# Autodesk Inventor assembly: ArmPower
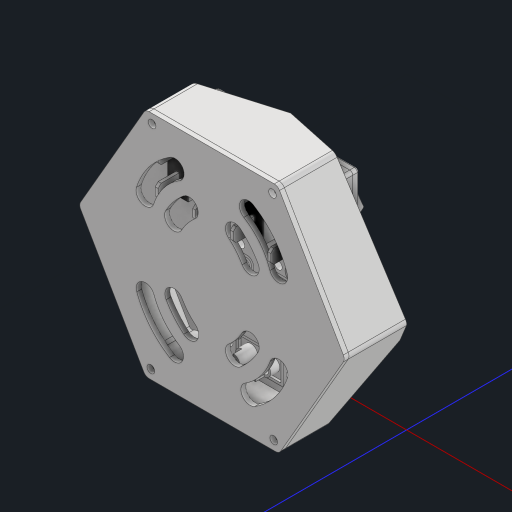
[picture p0: Inventor's stored thumbnail of the model, 512x512]
Saved by Autodesk Inventor 2023 (Build 270158000, 158)
## iProperties
Created: 2023-12-09
Part Number: ArmPower
Document SubType Name: Assembly
Designer: valer
Author: valer
## Documents named in this file (5)
- C:\Users\valer\Desktop\str1ker\cad\ArmPower.iam
- C:\Users\valer\Desktop\str1ker\cad\ArmPowerBoardWithControls.ipt
- C:\Users\valer\Desktop\str1ker\cad\ArmPowerBoardWithControlsLid.ipt
- C:\Users\valer\Desktop\str1ker\cad\external\XT-60EW-M.ipt
- C:\Users\valer\Desktop\str1ker\cad\external\ESwitchRD1.ipt
## Components (11 placed, 4 different names)
1. ArmPowerBoardWithControls:1 — Mate:1, Mate:2, Mate:3, Mate:4, Mate:5, Mate:6, Mate:7, Mate:8, Mate:9, Mate:10, Mate:11, Mate:12, Mate:13, Mate:14, Mate:15, Mate:16, Mate:17, Mate:18, Mate:19, Mate:20, Mate:21, Mate:22, Mate:23, Mate:24, Mate:25, Mate:26, Mate:27
2. ArmPowerBoardWithControlsLid:1 — Mate:1, Mate:2, Mate:3
3. XT-60EW-M:1 — Mate:4, Mate:5, Mate:6, Flush:1
4. ESwitchRD1:1 — Mate:7, Mate:8, Mate:9
5. ESwitchRD1:2 — Mate:10, Mate:11, Mate:12
6. ESwitchRD1:3 — Mate:13, Mate:14, Mate:15
7. ESwitchRD1:4 — Mate:16, Mate:17, Mate:18
8. XT-60EW-M:2 — Mate:19, Mate:20, Flush:1, Flush:2
9. XT-60EW-M:3 — Mate:21, Mate:22, Flush:2, Flush:3
10. XT-60EW-M:4 — Mate:25, Mate:26, Mate:27
11. XT-60EW-M:5 — Mate:23, Mate:24, Flush:3
## Relationships (30: Mate 27, Flush 3)
- Mate:1: ArmPowerBoardWithControls:1 ↔ ArmPowerBoardWithControlsLid:1
- Mate:2: ArmPowerBoardWithControls:1 ↔ ArmPowerBoardWithControlsLid:1
- Mate:3: ArmPowerBoardWithControls:1 ↔ ArmPowerBoardWithControlsLid:1
- Mate:4: ArmPowerBoardWithControls:1 ↔ XT-60EW-M:1
- Mate:5: ArmPowerBoardWithControls:1 ↔ XT-60EW-M:1
- Mate:6: ArmPowerBoardWithControls:1 ↔ XT-60EW-M:1
- Mate:7: ArmPowerBoardWithControls:1 ↔ ESwitchRD1:1
- Mate:8: ArmPowerBoardWithControls:1 ↔ ESwitchRD1:1
- Mate:9: ArmPowerBoardWithControls:1 ↔ ESwitchRD1:1
- Mate:10: ArmPowerBoardWithControls:1 ↔ ESwitchRD1:2
- Mate:11: ArmPowerBoardWithControls:1 ↔ ESwitchRD1:2
- Mate:12: ArmPowerBoardWithControls:1 ↔ ESwitchRD1:2
- Mate:13: ArmPowerBoardWithControls:1 ↔ ESwitchRD1:3
- Mate:14: ArmPowerBoardWithControls:1 ↔ ESwitchRD1:3
- Mate:15: ArmPowerBoardWithControls:1 ↔ ESwitchRD1:3
- Mate:16: ArmPowerBoardWithControls:1 ↔ ESwitchRD1:4
- Mate:17: ArmPowerBoardWithControls:1 ↔ ESwitchRD1:4
- Mate:18: ArmPowerBoardWithControls:1 ↔ ESwitchRD1:4
- Mate:19: ArmPowerBoardWithControls:1 ↔ XT-60EW-M:2
- Mate:20: ArmPowerBoardWithControls:1 ↔ XT-60EW-M:2
- Flush:1: XT-60EW-M:1 ↔ XT-60EW-M:2
- Mate:21: ArmPowerBoardWithControls:1 ↔ XT-60EW-M:3
- Mate:22: ArmPowerBoardWithControls:1 ↔ XT-60EW-M:3
- Flush:2: XT-60EW-M:2 ↔ XT-60EW-M:3
- Mate:23: ArmPowerBoardWithControls:1 ↔ XT-60EW-M:5
- Mate:24: ArmPowerBoardWithControls:1 ↔ XT-60EW-M:5
- Flush:3: XT-60EW-M:3 ↔ XT-60EW-M:5
- Mate:25: ArmPowerBoardWithControls:1 ↔ XT-60EW-M:4
- Mate:26: ArmPowerBoardWithControls:1 ↔ XT-60EW-M:4
- Mate:27: ArmPowerBoardWithControls:1 ↔ XT-60EW-M:4
